# Autodesk Inventor assembly: sedinetcam
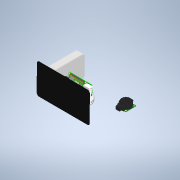
[picture p0: Inventor's stored thumbnail of the model, 180x180]
Saved by Autodesk Inventor 2021 (Build 250183000, 183)
## iProperties
Created: 2021-05-26
Part Number: sedinetcam
Document SubType Name: Assembly
Designer: jbs2071
Author: jbs2071
## Documents named in this file (7)
- C:\Users\jbs2071\SynologyDrive\MyDrive\SediNetCam\inventor\sedinetcam.iam
- C:\Users\jbs2071\SynologyDrive\MyDrive\SediNetCam\inventor\ringlight.ipt
- C:\Users\jbs2071\SynologyDrive\MyDrive\SediNetCam\inventor\v50battery.ipt
- C:\Users\jbs2071\SynologyDrive\MyDrive\SediNetCam\inventor\Raspberry Pi HQ Camera.ipt
- C:\Users\jbs2071\SynologyDrive\MyDrive\SediNetCam\inventor\Raspberry pi 4\Raspberry Pi 4 Model B.iam
- C:\Users\jbs2071\SynologyDrive\MyDrive\SediNetCam\inventor\lcd\raspberry pi display.iam
- C:\Users\jbs2071\SynologyDrive\MyDrive\SediNetCam\inventor\BerryIMU\BerryGPS-IMU-v4-step.ipt
## Components (6 placed, 6 different names)
1. ringlight:1
2. v50battery:1 — Mate:2
3. Raspberry Pi HQ Camera:1
4. Raspberry Pi 4 Model B:1 [sub-assembly] — Flush:1, Flush:2, Flush:3, Flush:4, Mate:3, Mate:4
5. raspberry pi display:1 [sub-assembly] — Flush:3, Flush:4, Mate:2, Mate:3
6. BerryGPS-IMU-v4-step:1 — Flush:1, Flush:2, Mate:4
## Relationships (7: Flush 4, Mate 3)
- Flush:1: Raspberry Pi 4 Model B:1 ↔ BerryGPS-IMU-v4-step:1
- Flush:2: Raspberry Pi 4 Model B:1 ↔ BerryGPS-IMU-v4-step:1
- Flush:3: Raspberry Pi 4 Model B:1 ↔ raspberry pi display:1
- Flush:4: Raspberry Pi 4 Model B:1 ↔ raspberry pi display:1
- Mate:2: v50battery:1 ↔ raspberry pi display:1
- Mate:3 (36.65 mm): Raspberry Pi 4 Model B:1 ↔ raspberry pi display:1
- Mate:4 (25 mm): Raspberry Pi 4 Model B:1 ↔ BerryGPS-IMU-v4-step:1
